# Autodesk Inventor assembly: MotorAssembly
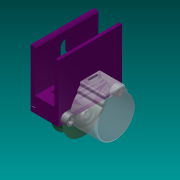
[picture p0: Inventor's stored thumbnail of the model, 180x180]
Saved by Autodesk Inventor 2013 (Build 170138000, 138)
## iProperties
Created: 2013-08-16
Part Number: MotorAssembly
Document SubType Name: Assembly
Designer: Sawaiz
Author: Sawaiz
## Documents named in this file (5)
- S:\Sawaiz\Documents\3D Modeling\Inventor\PolarGraph\MotorAssembly.iam
- S:\Sawaiz\Documents\3D Modeling\Inventor\PolarGraph\MotorClipV2.ipt
- S:\Sawaiz\Documents\3D Modeling\Inventor\PolarGraph\MotorFilamentSpool.iam
- S:\Sawaiz\Documents\3D Modeling\Inventor\PolarGraph\Imported Components\91841A009\91841A009.ipt
- S:\Sawaiz\Documents\3D Modeling\Inventor\Content Center Files\R2013\en-US\ANSI B18.3(05)\ANSI B18.3 - 8-32 UNC - 0.75(31).ipt
## Components (6 placed, 4 different names)
1. MotorClipV2:1 — Flush:1, Mate:7, Mate:8, Mate:9, Mate:10, Mate:11, Mate:12, Mate:13, Mate:14
2. MotorFilamentSpool:1 [sub-assembly] — Flush:1, Insert:1, Insert:2, Mate:7
3. 91841A009:2 — Mate:9, Mate:12, Mate:13
4. 91841A009:3 — Mate:10, Mate:11, Mate:14
5. Hexagon Socket Head Cap Screw - Inch No. 8 - 32 UNC - 3/4:1 — Insert:2
6. Hexagon Socket Head Cap Screw - Inch No. 8 - 32 UNC - 3/4:2 — Insert:1, Mate:8
## Relationships (11: Mate 8, Insert 2, Flush 1)
- Flush:1: MotorClipV2:1 ↔ MotorFilamentSpool:1
- Insert:1: MotorFilamentSpool:1 ↔ Hexagon Socket Head Cap Screw - Inch No. 8 - 32 UNC - 3/4:2
- Insert:2: MotorFilamentSpool:1 ↔ Hexagon Socket Head Cap Screw - Inch No. 8 - 32 UNC - 3/4:1
- Mate:7: MotorClipV2:1 ↔ MotorFilamentSpool:1
- Mate:8: MotorClipV2:1 ↔ Hexagon Socket Head Cap Screw - Inch No. 8 - 32 UNC - 3/4:2
- Mate:9: MotorClipV2:1 ↔ 91841A009:2
- Mate:10: MotorClipV2:1 ↔ 91841A009:3
- Mate:11: MotorClipV2:1 ↔ 91841A009:3
- Mate:12: MotorClipV2:1 ↔ 91841A009:2
- Mate:13: MotorClipV2:1 ↔ 91841A009:2
- Mate:14: MotorClipV2:1 ↔ 91841A009:3
